# Autodesk Inventor assembly: Swirly Assembly
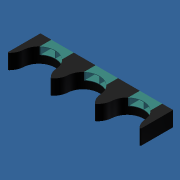
[picture p0: Inventor's stored thumbnail of the model, 180x180]
Saved by Autodesk Inventor 2012 (Build 160160000, 160)
## iProperties
Created: 2012-02-08
Part Number: Swirly Assembly
Document SubType Name: Assembly
Designer: Allison Garza
Author: Allison Garza
## Documents named in this file (3)
- C:\Users\Allison Garza\Documents\Rice Spring 2012\MRSL\Swirly Assembly.iam
- C:\Users\Allison Garza\Documents\Rice Spring 2012\MRSL\swirvy.ipt
- C:\Users\Allison Garza\Documents\Rice Spring 2012\MRSL\IR Sensor Piece.ipt
## Components (4 placed, 2 different names)
1. swirvy:1 — Mate:1, Mate:2, Flush:1, Mate:3, Mate:4, Mate:5, Mate:6, Flush:2, Flush:3
2. IR Sensor Piece:1 — Mate:1, Mate:2, Flush:1
3. IR Sensor Piece:2 — Mate:3, Mate:4, Flush:2
4. IR Sensor Piece:3 — Mate:5, Mate:6, Flush:3
## Relationships (9: Mate 6, Flush 3)
- Mate:1: swirvy:1 ↔ IR Sensor Piece:1
- Mate:2: swirvy:1 ↔ IR Sensor Piece:1
- Flush:1: swirvy:1 ↔ IR Sensor Piece:1
- Mate:3: swirvy:1 ↔ IR Sensor Piece:2
- Mate:4: swirvy:1 ↔ IR Sensor Piece:2
- Mate:5: swirvy:1 ↔ IR Sensor Piece:3
- Mate:6: swirvy:1 ↔ IR Sensor Piece:3
- Flush:2: swirvy:1 ↔ IR Sensor Piece:2
- Flush:3: swirvy:1 ↔ IR Sensor Piece:3
